# Autodesk Inventor assembly: Link3
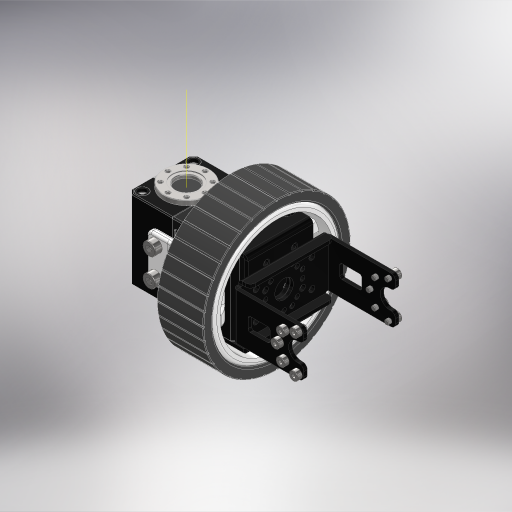
[picture p0: Inventor's stored thumbnail of the model, 512x512]
Saved by Autodesk Inventor 2023 (Build 270158000, 158)
## iProperties
Created: 2022-11-03
Part Number: Link3
Document SubType Name: Assembly
Designer: doore
Author: doore
## Documents named in this file (5)
- C:\Users\doore\OneDrive - 대구경북과학기술원\0.프로젝트\2019_뱀로봇\모델도면\MJC_정렬버전\Link3.iam
- C:\Users\doore\OneDrive - 대구경북과학기술원\0.프로젝트\2019_뱀로봇\모델도면\MJC_정렬버전\Haed.iam
- C:\Users\doore\OneDrive - 대구경북과학기술원\0.프로젝트\2019_뱀로봇\모델도면\MJC_정렬버전\assets\xm430_frame.ipt
- C:\Users\doore\OneDrive - 대구경북과학기술원\0.프로젝트\2019_뱀로봇\모델도면\MJC_정렬버전\assets\xm430_hinge.ipt
- C:\Users\doore\OneDrive\문서\Inventor\Content Center Files\R2023\ko-KR\BS 4168(1)\BS 4168 - M2 x 3(1).ipt
## Components (13 placed, 4 different names)
1. Haed:1 [sub-assembly] — 강체:1
2. xm430_frame:1 — 강체:1, 강체:2
3. xm430_hinge:1 — 강체:2, 강체:3, 강체:4, 강체:5, 강체:6, 강체:7, 강체:8, 강체:9, 강체:10, 강체:11, 강체:12
4. BS 4168 : 부품 1 6각 소켓 머리 캡 나사 - 미터 M2 x 3:1 — 강체:4
5. BS 4168 : 부품 1 6각 소켓 머리 캡 나사 - 미터 M2 x 3:2 — 강체:7
6. BS 4168 : 부품 1 6각 소켓 머리 캡 나사 - 미터 M2 x 3:3 — 강체:6
7. BS 4168 : 부품 1 6각 소켓 머리 캡 나사 - 미터 M2 x 3:4 — 강체:5
8. BS 4168 : 부품 1 6각 소켓 머리 캡 나사 - 미터 M2 x 3:5 — 강체:3
9. BS 4168 : 부품 1 6각 소켓 머리 캡 나사 - 미터 M2 x 3:6 — 강체:9
10. BS 4168 : 부품 1 6각 소켓 머리 캡 나사 - 미터 M2 x 3:7 — 강체:11
11. BS 4168 : 부품 1 6각 소켓 머리 캡 나사 - 미터 M2 x 3:8 — 강체:8
12. BS 4168 : 부품 1 6각 소켓 머리 캡 나사 - 미터 M2 x 3:9 — 강체:10
13. BS 4168 : 부품 1 6각 소켓 머리 캡 나사 - 미터 M2 x 3:10 — 강체:12
## Relationships (12: WeldJoint 12)
- 강체:1 [WeldJoint]: Haed:1 ↔ xm430_frame:1
- 강체:2 [WeldJoint]: xm430_frame:1 ↔ xm430_hinge:1
- 강체:3 [WeldJoint]: xm430_hinge:1 ↔ BS 4168 : 부품 1 6각 소켓 머리 캡 나사 - 미터 M2 x 3:5
- 강체:4 [WeldJoint]: xm430_hinge:1 ↔ BS 4168 : 부품 1 6각 소켓 머리 캡 나사 - 미터 M2 x 3:1
- 강체:5 [WeldJoint]: xm430_hinge:1 ↔ BS 4168 : 부품 1 6각 소켓 머리 캡 나사 - 미터 M2 x 3:4
- 강체:6 [WeldJoint]: xm430_hinge:1 ↔ BS 4168 : 부품 1 6각 소켓 머리 캡 나사 - 미터 M2 x 3:3
- 강체:7 [WeldJoint]: xm430_hinge:1 ↔ BS 4168 : 부품 1 6각 소켓 머리 캡 나사 - 미터 M2 x 3:2
- 강체:8 [WeldJoint]: xm430_hinge:1 ↔ BS 4168 : 부품 1 6각 소켓 머리 캡 나사 - 미터 M2 x 3:8
- 강체:9 [WeldJoint]: xm430_hinge:1 ↔ BS 4168 : 부품 1 6각 소켓 머리 캡 나사 - 미터 M2 x 3:6
- 강체:10 [WeldJoint]: xm430_hinge:1 ↔ BS 4168 : 부품 1 6각 소켓 머리 캡 나사 - 미터 M2 x 3:9
- 강체:11 [WeldJoint]: xm430_hinge:1 ↔ BS 4168 : 부품 1 6각 소켓 머리 캡 나사 - 미터 M2 x 3:7
- 강체:12 [WeldJoint]: xm430_hinge:1 ↔ BS 4168 : 부품 1 6각 소켓 머리 캡 나사 - 미터 M2 x 3:10
